# Autodesk Inventor assembly: Body
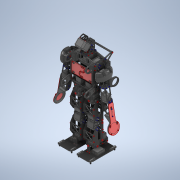
[picture p0: Inventor's stored thumbnail of the model, 180x180]
Saved by Autodesk Inventor 2022 (Build 260153000, 153)
## iProperties
Created: 2021-10-01
Part Number: Body
Document SubType Name: Assembly
Designer: Masato Kubotera
Mass: 3701.21 g
Surface Area: 13379.4 cm^2
Volume: 3277.75 cm^3
Author: Masato Kubotera
## Documents named in this file (5)
- C:\Users\MasatoKubotera\Desktop\SUSTAINA-OP\Body.iam
- C:\Users\MasatoKubotera\Documents\Inventor\SUSTAINA-OP\UpperBody\UpperBody.iam
- C:\Users\MasatoKubotera\Documents\Inventor\SUSTAINA-OP\LowerBody\LowerBody.iam
- C:\Users\MasatoKubotera\Documents\Inventor\SUSTAINA-OP\LowerBody\LowerBody_MIR.iam
- C:\Users\MasatoKubotera\Documents\Inventor\SUSTAINA-OP\Body.iam
## Components (3 placed, 3 different names)
1. UpperBody:1 [sub-assembly] — 挿入:1, 挿入:2, 角度:1, 角度:2, フラッシュ:1, フラッシュ:2
2. LowerBody:1 [sub-assembly] — 挿入:1, 角度:2, メイト:1
3. LowerBody_MIR:1 [sub-assembly] — 挿入:2, 角度:1
## Relationships (7: Insert 2, Angle 2, Flush 2, Mate 1)
- 挿入:1 [Insert]: UpperBody:1 ↔ LowerBody:1
- 挿入:2 [Insert]: UpperBody:1 ↔ LowerBody_MIR:1
- 角度:1 [Angle] (0 deg): UpperBody:1 ↔ LowerBody_MIR:1
- 角度:2 [Angle] (0 deg): UpperBody:1 ↔ LowerBody:1
- フラッシュ:1 [Flush]: UpperBody:1
- フラッシュ:2 [Flush]: UpperBody:1
- メイト:1 [Mate]: LowerBody:1
